# Autodesk Inventor assembly: CathodeCage
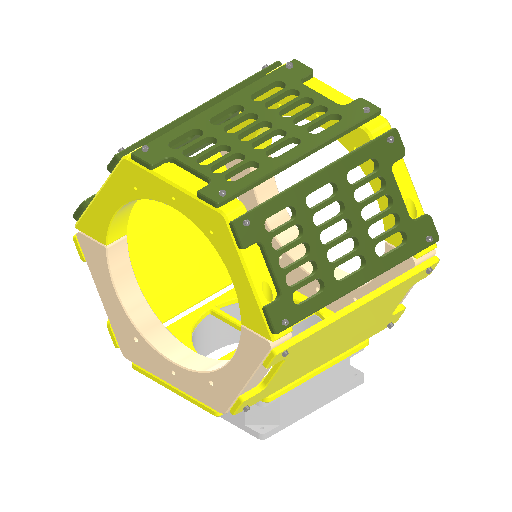
[picture p0: Inventor's stored thumbnail of the model, 512x512]
Saved by Autodesk Inventor 2026.2 (Build 302298000, 298)
## iProperties
Created: 2023-12-04
Part Number: CathodeCage
Document SubType Name: Assembly
Designer: kuzmin
Author: kuzmin
## Documents named in this file (11)
- D:\repos\PIHTI\Plasma Vessel\Cathode-Flange-Cage\CathodeCage.iam
- D:\repos\PIHTI\Plasma Vessel\Cathode-Flange-Cage\Baseplate-for-ICF152-flange-outer-part.ipt
- D:\repos\PIHTI\Plasma Vessel\Cathode-Flange-Cage\Cathode-Cover-Plate.ipt
- D:\repos\PIHTI\Plasma Vessel\Cathode-Flange-Cage\AC-fan-case.ipt
- D:\repos\PIHTI\Plasma Vessel\Cathode-Flange-Cage\Cathode-Cover-Plate-top-side-front.ipt
- D:\repos\PIHTI\Plasma Vessel\Cathode-Flange-Cage\Cathode-Cover-Plate-bottom-side.ipt
- D:\repos\PIHTI\Plasma Vessel\Cathode-Flange-Cage\Baseplate-for-ICF152-flange-outer-part-bottom.ipt
- D:\repos\PIHTI\ContentCenter\Fastners\M4-nut.ipt
- D:\repos\PIHTI\ContentCenter\Fastners\M4x30-SHCS.ipt
- D:\repos\PIHTI\ContentCenter\Fastners\M3x10-SHCS.ipt
- D:\repos\PIHTI\ContentCenter\Fastners\brass-insert-m3x5.ipt
## Components (57 placed, 10 different names)
1. Baseplate-for-ICF152-flange-outer-part:1 — メイト:5, メイト:6, メイト:7, メイト:13, メイト:14, メイト:22, メイト:23, メイト:38, 回転:4, 回転:5, リジッド:10, リジッド:40
2. Baseplate-for-ICF152-flange-outer-part:3 — メイト:3, メイト:4, メイト:8, メイト:21, メイト:24, 回転:6, 回転:7
3. Cathode-Cover-Plate:1 — メイト:28, メイト:29, メイト:30, メイト:32, メイト:35, 回転:24, 回転:25, 回転:26, 回転:27, メイト:39
4. AC-fan-case:1 — メイト:28, メイト:29, メイト:30
5. Cathode-Cover-Plate-top-side-front:1 — メイト:13, メイト:21, メイト:22, 回転:12, 回転:13, 回転:14, 回転:15
6. Cathode-Cover-Plate-top-side-front:2 — メイト:14, メイト:23, メイト:24, 回転:16, 回転:17, 回転:18, 回転:19
7. Cathode-Cover-Plate-top-side-front:3 — メイト:3, メイト:4, メイト:5, メイト:6, メイト:7, メイト:8, 回転:8, 回転:9, 回転:10, 回転:11
8. Cathode-Cover-Plate-bottom-side:1 — 回転:28, 回転:29, 回転:30, 回転:31, リジッド:50
9. Cathode-Cover-Plate-bottom-side:2 — 回転:20, 回転:21, 回転:22, 回転:23, リジッド:45
10. Baseplate-for-ICF152-flange-outer-part-bottom:1 — メイト:32, メイト:39, メイト:42, 回転:34, 回転:35, リジッド:43, リジッド:44, リジッド:46, リジッド:47, 回転:38, リジッド:51
11. Baseplate-for-ICF152-flange-outer-part-bottom:2 — メイト:35, メイト:38, メイト:40, メイト:41, メイト:44, リジッド:6, リジッド:7, リジッド:39, リジッド:40, リジッド:41, リジッド:42, リジッド:45, リジッド:48, 回転:36, リジッド:49, リジッド:50
12. JIS B 1176 - Metric M3 x 10:1 — 回転:22
13. JIS B 1176 - Metric M3 x 10:2 — 回転:21, メイト:44
14. JIS B 1176 - Metric M3 x 10:3 — 回転:20
15. JIS B 1176 - Metric M3 x 10:4 — 回転:8
16. JIS B 1176 - Metric M3 x 10:5 — 回転:27
17. JIS B 1176 - Metric M3 x 10:6 — 回転:26, メイト:40
18. JIS B 1176 - Metric M3 x 10:7 — 回転:25
19. JIS B 1176 - Metric M3 x 10:8 — 回転:24
20. JIS B 1176 - Metric M3 x 10:9 — 回転:28, メイト:41
21. JIS B 1176 - Metric M3 x 10:10 — 回転:29
22. JIS B 1176 - Metric M3 x 10:11 — 回転:30, メイト:42
23. JIS B 1176 - Metric M3 x 10:12 — 回転:31
24. JIS B 1176 - Metric M3 x 10:13 — 回転:14
25. JIS B 1176 - Metric M3 x 10:14 — 回転:15
26. JIS B 1176 - Metric M3 x 10:15 — 回転:23
27. JIS B 1176 - Metric M3 x 10:16 — 回転:13
28. JIS B 1176 - Metric M3 x 10:17 — 回転:9
29. JIS B 1176 - Metric M3 x 10:18 — 回転:10
30. JIS B 1176 - Metric M3 x 10:19 — 回転:11
31. JIS B 1176 - Metric M3 x 10:20 — 回転:12
32. JIS B 1176 - Metric M3 x 10:21 — 回転:16
33. JIS B 1176 - Metric M3 x 10:22 — 回転:17
34. JIS B 1176 - Metric M3 x 10:23 — 回転:18
35. JIS B 1176 - Metric M3 x 10:24 — 回転:19
36. JIS B 1181 -finished Class 1 - Metric Class 1 -finishedM4:1
37. JIS B 1181 -finished Class 1 - Metric Class 1 -finishedM4:2 — 回転:38
38. JIS B 1181 -finished Class 1 - Metric Class 1 -finishedM4:3 — リジッド:49
39. JIS B 1181 -finished Class 1 - Metric Class 1 -finishedM4:4 — リジッド:51
40. JIS B 1176 - Metric M4 x 30:1 — 回転:7
41. JIS B 1176 - Metric M4 x 30:2 — 回転:6
42. JIS B 1176 - Metric M4 x 30:3 — 回転:5
43. JIS B 1176 - Metric M4 x 30:4 — 回転:4
44. brass-insert-m3x5:1 — リジッド:46
45. brass-insert-m3x5:2 — リジッド:47
46. brass-insert-m3x5:3 — 回転:35
47. brass-insert-m3x5:4 — 回転:34
48. brass-insert-m3x5:5 — リジッド:44
49. brass-insert-m3x5:6 — リジッド:43
50. brass-insert-m3x5:7 — リジッド:42
51. brass-insert-m3x5:8 — リジッド:6
52. brass-insert-m3x5:9 — リジッド:41
53. brass-insert-m3x5:10 — リジッド:7
54. brass-insert-m3x5:11 — 回転:36
55. brass-insert-m3x5:12 — リジッド:48
56. brass-insert-m3x5:13 — リジッド:10
57. brass-insert-m3x5:14 — リジッド:39
## Relationships (71: RevoluteJoint 32, Mate 23, WeldJoint 16)
- メイト:3 [Mate]: Baseplate-for-ICF152-flange-outer-part:3 ↔ Cathode-Cover-Plate-top-side-front:3
- メイト:4 [Mate]: Baseplate-for-ICF152-flange-outer-part:3 ↔ Cathode-Cover-Plate-top-side-front:3
- メイト:5 [Mate]: Baseplate-for-ICF152-flange-outer-part:1 ↔ Cathode-Cover-Plate-top-side-front:3
- メイト:6 [Mate]: Baseplate-for-ICF152-flange-outer-part:1 ↔ Cathode-Cover-Plate-top-side-front:3
- メイト:7 [Mate]: Baseplate-for-ICF152-flange-outer-part:1 ↔ Cathode-Cover-Plate-top-side-front:3
- メイト:8 [Mate]: Baseplate-for-ICF152-flange-outer-part:3 ↔ Cathode-Cover-Plate-top-side-front:3
- メイト:13 [Mate]: Baseplate-for-ICF152-flange-outer-part:1 ↔ Cathode-Cover-Plate-top-side-front:1
- メイト:14 [Mate]: Baseplate-for-ICF152-flange-outer-part:1 ↔ Cathode-Cover-Plate-top-side-front:2
- メイト:21 [Mate]: Baseplate-for-ICF152-flange-outer-part:3 ↔ Cathode-Cover-Plate-top-side-front:1
- メイト:22 [Mate]: Baseplate-for-ICF152-flange-outer-part:1 ↔ Cathode-Cover-Plate-top-side-front:1
- メイト:23 [Mate]: Baseplate-for-ICF152-flange-outer-part:1 ↔ Cathode-Cover-Plate-top-side-front:2
- メイト:24 [Mate]: Baseplate-for-ICF152-flange-outer-part:3 ↔ Cathode-Cover-Plate-top-side-front:2
- メイト:28 [Mate]: Cathode-Cover-Plate:1 ↔ AC-fan-case:1
- メイト:29 [Mate]: Cathode-Cover-Plate:1 ↔ AC-fan-case:1
- メイト:30 [Mate] (-101 mm): Cathode-Cover-Plate:1 ↔ AC-fan-case:1
- メイト:32 [Mate]: Cathode-Cover-Plate:1 ↔ Baseplate-for-ICF152-flange-outer-part-bottom:1
- メイト:35 [Mate]: Cathode-Cover-Plate:1 ↔ Baseplate-for-ICF152-flange-outer-part-bottom:2
- メイト:38 [Mate]: Baseplate-for-ICF152-flange-outer-part:1 ↔ Baseplate-for-ICF152-flange-outer-part-bottom:2
- 回転:4 [RevoluteJoint]: Baseplate-for-ICF152-flange-outer-part:1 ↔ JIS B 1176 - Metric M4 x 30:4
- 回転:5 [RevoluteJoint]: Baseplate-for-ICF152-flange-outer-part:1 ↔ JIS B 1176 - Metric M4 x 30:3
- 回転:6 [RevoluteJoint]: Baseplate-for-ICF152-flange-outer-part:3 ↔ JIS B 1176 - Metric M4 x 30:2
- 回転:7 [RevoluteJoint]: Baseplate-for-ICF152-flange-outer-part:3 ↔ JIS B 1176 - Metric M4 x 30:1
- 回転:8 [RevoluteJoint]: Cathode-Cover-Plate-top-side-front:3 ↔ JIS B 1176 - Metric M3 x 10:4
- 回転:9 [RevoluteJoint]: Cathode-Cover-Plate-top-side-front:3 ↔ JIS B 1176 - Metric M3 x 10:17
- 回転:10 [RevoluteJoint]: Cathode-Cover-Plate-top-side-front:3 ↔ JIS B 1176 - Metric M3 x 10:18
- 回転:11 [RevoluteJoint]: Cathode-Cover-Plate-top-side-front:3 ↔ JIS B 1176 - Metric M3 x 10:19
- 回転:12 [RevoluteJoint]: Cathode-Cover-Plate-top-side-front:1 ↔ JIS B 1176 - Metric M3 x 10:20
- 回転:13 [RevoluteJoint]: Cathode-Cover-Plate-top-side-front:1 ↔ JIS B 1176 - Metric M3 x 10:16
- 回転:14 [RevoluteJoint]: Cathode-Cover-Plate-top-side-front:1 ↔ JIS B 1176 - Metric M3 x 10:13
- 回転:15 [RevoluteJoint]: Cathode-Cover-Plate-top-side-front:1 ↔ JIS B 1176 - Metric M3 x 10:14
- 回転:16 [RevoluteJoint]: Cathode-Cover-Plate-top-side-front:2 ↔ JIS B 1176 - Metric M3 x 10:21
- 回転:17 [RevoluteJoint]: Cathode-Cover-Plate-top-side-front:2 ↔ JIS B 1176 - Metric M3 x 10:22
- 回転:18 [RevoluteJoint]: Cathode-Cover-Plate-top-side-front:2 ↔ JIS B 1176 - Metric M3 x 10:23
- 回転:19 [RevoluteJoint]: Cathode-Cover-Plate-top-side-front:2 ↔ JIS B 1176 - Metric M3 x 10:24
- 回転:20 [RevoluteJoint]: Cathode-Cover-Plate-bottom-side:2 ↔ JIS B 1176 - Metric M3 x 10:3
- 回転:21 [RevoluteJoint]: Cathode-Cover-Plate-bottom-side:2 ↔ JIS B 1176 - Metric M3 x 10:2
- 回転:22 [RevoluteJoint]: Cathode-Cover-Plate-bottom-side:2 ↔ JIS B 1176 - Metric M3 x 10:1
- 回転:23 [RevoluteJoint]: Cathode-Cover-Plate-bottom-side:2 ↔ JIS B 1176 - Metric M3 x 10:15
- 回転:24 [RevoluteJoint]: Cathode-Cover-Plate:1 ↔ JIS B 1176 - Metric M3 x 10:8
- 回転:25 [RevoluteJoint]: Cathode-Cover-Plate:1 ↔ JIS B 1176 - Metric M3 x 10:7
- 回転:26 [RevoluteJoint]: Cathode-Cover-Plate:1 ↔ JIS B 1176 - Metric M3 x 10:6
- 回転:27 [RevoluteJoint]: Cathode-Cover-Plate:1 ↔ JIS B 1176 - Metric M3 x 10:5
- 回転:28 [RevoluteJoint]: Cathode-Cover-Plate-bottom-side:1 ↔ JIS B 1176 - Metric M3 x 10:9
- 回転:29 [RevoluteJoint]: Cathode-Cover-Plate-bottom-side:1 ↔ JIS B 1176 - Metric M3 x 10:10
- 回転:30 [RevoluteJoint]: Cathode-Cover-Plate-bottom-side:1 ↔ JIS B 1176 - Metric M3 x 10:11
- 回転:31 [RevoluteJoint]: Cathode-Cover-Plate-bottom-side:1 ↔ JIS B 1176 - Metric M3 x 10:12
- メイト:39 [Mate]: Cathode-Cover-Plate:1 ↔ Baseplate-for-ICF152-flange-outer-part-bottom:1
- メイト:40 [Mate]: Baseplate-for-ICF152-flange-outer-part-bottom:2 ↔ JIS B 1176 - Metric M3 x 10:6
- メイト:41 [Mate]: Baseplate-for-ICF152-flange-outer-part-bottom:2 ↔ JIS B 1176 - Metric M3 x 10:9
- メイト:42 [Mate]: Baseplate-for-ICF152-flange-outer-part-bottom:1 ↔ JIS B 1176 - Metric M3 x 10:11
- メイト:44 [Mate]: Baseplate-for-ICF152-flange-outer-part-bottom:2 ↔ JIS B 1176 - Metric M3 x 10:2
- リジッド:6 [WeldJoint]: Baseplate-for-ICF152-flange-outer-part-bottom:2 ↔ brass-insert-m3x5:8
- リジッド:7 [WeldJoint]: Baseplate-for-ICF152-flange-outer-part-bottom:2 ↔ brass-insert-m3x5:10
- 回転:34 [RevoluteJoint]: Baseplate-for-ICF152-flange-outer-part-bottom:1 ↔ brass-insert-m3x5:4
- 回転:35 [RevoluteJoint]: Baseplate-for-ICF152-flange-outer-part-bottom:1 ↔ brass-insert-m3x5:3
- リジッド:39 [WeldJoint]: Baseplate-for-ICF152-flange-outer-part-bottom:2 ↔ brass-insert-m3x5:14
- リジッド:10 [WeldJoint]: Baseplate-for-ICF152-flange-outer-part:1 ↔ brass-insert-m3x5:13
- リジッド:40 [WeldJoint]: Baseplate-for-ICF152-flange-outer-part:1 ↔ Baseplate-for-ICF152-flange-outer-part-bottom:2
- リジッド:41 [WeldJoint]: Baseplate-for-ICF152-flange-outer-part-bottom:2 ↔ brass-insert-m3x5:9
- リジッド:42 [WeldJoint]: Baseplate-for-ICF152-flange-outer-part-bottom:2 ↔ brass-insert-m3x5:7
- リジッド:43 [WeldJoint]: Baseplate-for-ICF152-flange-outer-part-bottom:1 ↔ brass-insert-m3x5:6
- リジッド:44 [WeldJoint]: Baseplate-for-ICF152-flange-outer-part-bottom:1 ↔ brass-insert-m3x5:5
- リジッド:45 [WeldJoint]: Cathode-Cover-Plate-bottom-side:2 ↔ Baseplate-for-ICF152-flange-outer-part-bottom:2
- リジッド:46 [WeldJoint]: Baseplate-for-ICF152-flange-outer-part-bottom:1 ↔ brass-insert-m3x5:1
- リジッド:47 [WeldJoint]: Baseplate-for-ICF152-flange-outer-part-bottom:1 ↔ brass-insert-m3x5:2
- リジッド:48 [WeldJoint]: Baseplate-for-ICF152-flange-outer-part-bottom:2 ↔ brass-insert-m3x5:12
- 回転:36 [RevoluteJoint]: Baseplate-for-ICF152-flange-outer-part-bottom:2 ↔ brass-insert-m3x5:11
- リジッド:49 [WeldJoint]: Baseplate-for-ICF152-flange-outer-part-bottom:2 ↔ JIS B 1181 -finished Class 1 - Metric Class 1 -finishedM4:3
- 回転:38 [RevoluteJoint]: Baseplate-for-ICF152-flange-outer-part-bottom:1 ↔ JIS B 1181 -finished Class 1 - Metric Class 1 -finishedM4:2
- リジッド:50 [WeldJoint]: Cathode-Cover-Plate-bottom-side:1 ↔ Baseplate-for-ICF152-flange-outer-part-bottom:2
- リジッド:51 [WeldJoint]: Baseplate-for-ICF152-flange-outer-part-bottom:1 ↔ JIS B 1181 -finished Class 1 - Metric Class 1 -finishedM4:4
